# Autodesk Inventor assembly: Общая сборка
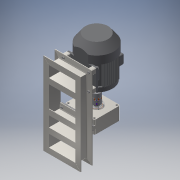
[picture p0: Inventor's stored thumbnail of the model, 180x180]
Saved by Autodesk Inventor 2016 (Build 200138000, 138)
## iProperties
Created: 2021-04-30
Part Number: Общая сборка
Material: Типовые
Document SubType Name: Assembly
Designer: Лол
Author: Лол
## Documents named in this file (11)
- C:\Users\Лол\Documents\Inventor\course_work\Общая сборка.iam
- C:\Users\Лол\Documents\Inventor\course_work\Муфта двигателя.iam
- C:\Users\Лол\Documents\Inventor\course_work\Электродвигатель АИР132S4,6,8.ipt
- C:\Users\Лол\Documents\Inventor\course_work\Редуктор.iam
- C:\Users\Лол\Documents\Inventor\course_work\Рама_02.iam
- C:\Users\Лол\Documents\Inventor\course_work\Болт 2 M12×30 ГОСТ 15591-70.ipt
- C:\Users\Лол\Documents\Inventor\course_work\Шайба 2 12Л ГОСТ 6402-78.ipt
- C:\Users\Лол\Documents\Inventor\course_work\Гайка M12-6H ГОСТ 5927-70.ipt
- C:\Users\Лол\Documents\Inventor\course_work\Болт 2 M12×70 ГОСТ 15591-70.ipt
- C:\Users\Лол\Documents\Inventor\course_work\Муфта 30мм.iam
- C:\Users\Лол\Documents\Inventor\course_work\AS 1421 - M8x16 конический.ipt
## Components (31 placed, 10 different names)
1. Муфта двигателя:1 [sub-assembly] — Совмещение:1, Совмещение:2, Совмещение:3, Совмещение:4, Заподлицо:1
2. Электродвигатель АИР132S4,6,8:1 — Совмещение:1, Совмещение:2, Совмещение:3, Угол:1, Совмещение:8, Совмещение:9, Совмещение:26, Совмещение:39, Совмещение:41, Совмещение:43
3. Редуктор:1 [sub-assembly] — Совмещение:4, Угол:1, Заподлицо:1, Совмещение:7, Совмещение:19, Совмещение:51, Совмещение:55, Совмещение:56, Совмещение:63, Совмещение:64, Совмещение:65, Совмещение:67
4. Рама_02:1 [sub-assembly] — Совмещение:7, Совмещение:8, Совмещение:9, Совмещение:10, Совмещение:11, Совмещение:12, Совмещение:13, Совмещение:14, Совмещение:15, Совмещение:16, Совмещение:17, Совмещение:23, Совмещение:24, Совмещение:29, Совмещение:30, Заподлицо:2, Совмещение:32, Совмещение:33, Совмещение:34, Совмещение:35, Совмещение:36, Совмещение:37
5. Болт 2 M12×30 ГОСТ 15591-70:1 — Совмещение:15, Совмещение:17, Совмещение:54, Совмещение:61
6. Болт 2 M12×30 ГОСТ 15591-70:2 — Совмещение:14, Совмещение:16, Совмещение:57, Совмещение:59
7. Болт 2 M12×30 ГОСТ 15591-70:3 — Совмещение:11, Совмещение:13, Совмещение:18, Совмещение:20
8. Болт 2 M12×30 ГОСТ 15591-70:4 — Совмещение:10, Совмещение:12, Совмещение:50, Совмещение:52
9. Шайба 2 12Л ГОСТ 6402-78:1 — Совмещение:25, Совмещение:26, Совмещение:28
10. Шайба 2 12Л ГОСТ 6402-78:4 — Совмещение:18, Совмещение:19, Совмещение:31
11. Гайка M12-6H ГОСТ 5927-70:1 — Совмещение:20, Совмещение:31
12. Болт 2 M12×70 ГОСТ 15591-70:1 — Совмещение:23, Совмещение:24, Совмещение:25, Совмещение:27
13. Гайка M12-6H ГОСТ 5927-70:2 — Совмещение:27, Совмещение:28
14. Гайка M12-6H ГОСТ 5927-70:3 — Совмещение:59, Совмещение:60
15. Гайка M12-6H ГОСТ 5927-70:4 — Совмещение:44, Совмещение:45
16. Гайка M12-6H ГОСТ 5927-70:5 — Совмещение:48, Совмещение:49
17. Гайка M12-6H ГОСТ 5927-70:6 — Совмещение:46, Совмещение:47
18. Гайка M12-6H ГОСТ 5927-70:7 — Совмещение:52, Совмещение:53
19. Гайка M12-6H ГОСТ 5927-70:8 — Совмещение:61, Совмещение:62
20. Шайба 2 12Л ГОСТ 6402-78:5 — Совмещение:56, Совмещение:57, Совмещение:60
21. Шайба 2 12Л ГОСТ 6402-78:6 — Совмещение:40, Совмещение:41, Совмещение:45
22. Шайба 2 12Л ГОСТ 6402-78:7 — Совмещение:42, Совмещение:43, Совмещение:48
23. Шайба 2 12Л ГОСТ 6402-78:8 — Совмещение:38, Совмещение:39, Совмещение:46
24. Шайба 2 12Л ГОСТ 6402-78:9 — Совмещение:50, Совмещение:51, Совмещение:53
25. Шайба 2 12Л ГОСТ 6402-78:10 — Совмещение:54, Совмещение:55, Совмещение:62
26. Болт 2 M12×70 ГОСТ 15591-70:2 — Совмещение:34, Совмещение:35, Совмещение:38, Совмещение:47
27. Болт 2 M12×70 ГОСТ 15591-70:3 — Совмещение:32, Совмещение:33, Совмещение:40, Совмещение:44
28. Болт 2 M12×70 ГОСТ 15591-70:4 — Совмещение:36, Совмещение:37, Совмещение:42, Совмещение:49
29. Муфта 30мм:1 [sub-assembly] — Совмещение:63, Совмещение:64, Совмещение:65, Совмещение:66, Совмещение:68, Совмещение:69
30. AS 1421 - M8x16 конический:1 — Совмещение:66, Совмещение:67
31. AS 1421 - M8x16 конический:2 — Совмещение:68, Совмещение:69
## Relationships (67: Mate 64, Flush 2, Angle 1)
- Совмещение:1 [Mate]: Муфта двигателя:1 ↔ Электродвигатель АИР132S4,6,8:1
- Совмещение:2 [Mate]: Муфта двигателя:1 ↔ Электродвигатель АИР132S4,6,8:1
- Совмещение:3 [Mate] (-35 mm): Муфта двигателя:1 ↔ Электродвигатель АИР132S4,6,8:1
- Совмещение:4 [Mate]: Муфта двигателя:1 ↔ Редуктор:1
- Угол:1 [Angle] (0 deg): Электродвигатель АИР132S4,6,8:1 ↔ Редуктор:1
- Заподлицо:1 [Flush] (5 mm): Муфта двигателя:1 ↔ Редуктор:1
- Совмещение:7 [Mate] (10 mm): Редуктор:1 ↔ Рама_02:1
- Совмещение:8 [Mate]: Электродвигатель АИР132S4,6,8:1 ↔ Рама_02:1
- Совмещение:9 [Mate]: Электродвигатель АИР132S4,6,8:1 ↔ Рама_02:1
- Совмещение:10 [Mate]: Рама_02:1 ↔ Болт 2 M12×30 ГОСТ 15591-70:4
- Совмещение:11 [Mate]: Рама_02:1 ↔ Болт 2 M12×30 ГОСТ 15591-70:3
- Совмещение:12 [Mate]: Рама_02:1 ↔ Болт 2 M12×30 ГОСТ 15591-70:4
- Совмещение:13 [Mate]: Рама_02:1 ↔ Болт 2 M12×30 ГОСТ 15591-70:3
- Совмещение:14 [Mate]: Рама_02:1 ↔ Болт 2 M12×30 ГОСТ 15591-70:2
- Совмещение:15 [Mate]: Рама_02:1 ↔ Болт 2 M12×30 ГОСТ 15591-70:1
- Совмещение:16 [Mate]: Рама_02:1 ↔ Болт 2 M12×30 ГОСТ 15591-70:2
- Совмещение:17 [Mate]: Рама_02:1 ↔ Болт 2 M12×30 ГОСТ 15591-70:1
- Совмещение:18 [Mate]: Болт 2 M12×30 ГОСТ 15591-70:3 ↔ Шайба 2 12Л ГОСТ 6402-78:4
- Совмещение:19 [Mate]: Редуктор:1 ↔ Шайба 2 12Л ГОСТ 6402-78:4
- Совмещение:20 [Mate]: Болт 2 M12×30 ГОСТ 15591-70:3 ↔ Гайка M12-6H ГОСТ 5927-70:1
- Совмещение:23 [Mate]: Рама_02:1 ↔ Болт 2 M12×70 ГОСТ 15591-70:1
- Совмещение:24 [Mate]: Рама_02:1 ↔ Болт 2 M12×70 ГОСТ 15591-70:1
- Совмещение:25 [Mate]: Шайба 2 12Л ГОСТ 6402-78:1 ↔ Болт 2 M12×70 ГОСТ 15591-70:1
- Совмещение:26 [Mate]: Электродвигатель АИР132S4,6,8:1 ↔ Шайба 2 12Л ГОСТ 6402-78:1
- Совмещение:27 [Mate]: Болт 2 M12×70 ГОСТ 15591-70:1 ↔ Гайка M12-6H ГОСТ 5927-70:2
- Совмещение:28 [Mate]: Шайба 2 12Л ГОСТ 6402-78:1 ↔ Гайка M12-6H ГОСТ 5927-70:2
- Совмещение:29 [Mate]: Рама_02:1
- Совмещение:30 [Mate]: Рама_02:1
- Заподлицо:2 [Flush]: Рама_02:1
- Совмещение:31 [Mate]: Шайба 2 12Л ГОСТ 6402-78:4 ↔ Гайка M12-6H ГОСТ 5927-70:1
- Совмещение:32 [Mate]: Рама_02:1 ↔ Болт 2 M12×70 ГОСТ 15591-70:3
- Совмещение:33 [Mate]: Рама_02:1 ↔ Болт 2 M12×70 ГОСТ 15591-70:3
- Совмещение:34 [Mate]: Рама_02:1 ↔ Болт 2 M12×70 ГОСТ 15591-70:2
- Совмещение:35 [Mate]: Рама_02:1 ↔ Болт 2 M12×70 ГОСТ 15591-70:2
- Совмещение:36 [Mate]: Рама_02:1 ↔ Болт 2 M12×70 ГОСТ 15591-70:4
- Совмещение:37 [Mate]: Рама_02:1 ↔ Болт 2 M12×70 ГОСТ 15591-70:4
- Совмещение:38 [Mate]: Шайба 2 12Л ГОСТ 6402-78:8 ↔ Болт 2 M12×70 ГОСТ 15591-70:2
- Совмещение:39 [Mate]: Электродвигатель АИР132S4,6,8:1 ↔ Шайба 2 12Л ГОСТ 6402-78:8
- Совмещение:40 [Mate]: Шайба 2 12Л ГОСТ 6402-78:6 ↔ Болт 2 M12×70 ГОСТ 15591-70:3
- Совмещение:41 [Mate]: Электродвигатель АИР132S4,6,8:1 ↔ Шайба 2 12Л ГОСТ 6402-78:6
- Совмещение:42 [Mate]: Шайба 2 12Л ГОСТ 6402-78:7 ↔ Болт 2 M12×70 ГОСТ 15591-70:4
- Совмещение:43 [Mate]: Электродвигатель АИР132S4,6,8:1 ↔ Шайба 2 12Л ГОСТ 6402-78:7
- Совмещение:44 [Mate]: Гайка M12-6H ГОСТ 5927-70:4 ↔ Болт 2 M12×70 ГОСТ 15591-70:3
- Совмещение:45 [Mate]: Гайка M12-6H ГОСТ 5927-70:4 ↔ Шайба 2 12Л ГОСТ 6402-78:6
- Совмещение:46 [Mate]: Гайка M12-6H ГОСТ 5927-70:6 ↔ Шайба 2 12Л ГОСТ 6402-78:8
- Совмещение:47 [Mate]: Гайка M12-6H ГОСТ 5927-70:6 ↔ Болт 2 M12×70 ГОСТ 15591-70:2
- Совмещение:48 [Mate]: Гайка M12-6H ГОСТ 5927-70:5 ↔ Шайба 2 12Л ГОСТ 6402-78:7
- Совмещение:49 [Mate]: Гайка M12-6H ГОСТ 5927-70:5 ↔ Болт 2 M12×70 ГОСТ 15591-70:4
- Совмещение:50 [Mate]: Болт 2 M12×30 ГОСТ 15591-70:4 ↔ Шайба 2 12Л ГОСТ 6402-78:9
- Совмещение:51 [Mate]: Редуктор:1 ↔ Шайба 2 12Л ГОСТ 6402-78:9
- Совмещение:52 [Mate]: Болт 2 M12×30 ГОСТ 15591-70:4 ↔ Гайка M12-6H ГОСТ 5927-70:7
- Совмещение:53 [Mate]: Гайка M12-6H ГОСТ 5927-70:7 ↔ Шайба 2 12Л ГОСТ 6402-78:9
- Совмещение:54 [Mate]: Болт 2 M12×30 ГОСТ 15591-70:1 ↔ Шайба 2 12Л ГОСТ 6402-78:10
- Совмещение:55 [Mate]: Редуктор:1 ↔ Шайба 2 12Л ГОСТ 6402-78:10
- Совмещение:56 [Mate]: Редуктор:1 ↔ Шайба 2 12Л ГОСТ 6402-78:5
- Совмещение:57 [Mate]: Болт 2 M12×30 ГОСТ 15591-70:2 ↔ Шайба 2 12Л ГОСТ 6402-78:5
- Совмещение:59 [Mate]: Болт 2 M12×30 ГОСТ 15591-70:2 ↔ Гайка M12-6H ГОСТ 5927-70:3
- Совмещение:60 [Mate]: Гайка M12-6H ГОСТ 5927-70:3 ↔ Шайба 2 12Л ГОСТ 6402-78:5
- Совмещение:61 [Mate]: Болт 2 M12×30 ГОСТ 15591-70:1 ↔ Гайка M12-6H ГОСТ 5927-70:8
- Совмещение:62 [Mate]: Гайка M12-6H ГОСТ 5927-70:8 ↔ Шайба 2 12Л ГОСТ 6402-78:10
- Совмещение:63 [Mate]: Редуктор:1 ↔ Муфта 30мм:1
- Совмещение:64 [Mate]: Редуктор:1 ↔ Муфта 30мм:1
- Совмещение:65 [Mate] (-30 mm): Редуктор:1 ↔ Муфта 30мм:1
- Совмещение:66 [Mate]: Муфта 30мм:1 ↔ AS 1421 - M8x16 конический:1
- Совмещение:67 [Mate]: Редуктор:1 ↔ AS 1421 - M8x16 конический:1
- Совмещение:68 [Mate]: Муфта 30мм:1 ↔ AS 1421 - M8x16 конический:2
- Совмещение:69 [Mate]: Муфта 30мм:1 ↔ AS 1421 - M8x16 конический:2
